# Autodesk Inventor assembly: wheel90mmwithbearing_MIR
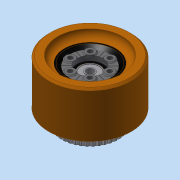
[picture p0: Inventor's stored thumbnail of the model, 180x180]
Saved by Autodesk Inventor 2014 SP1 (Build 180222100, 222)
## iProperties
Created: 2014-05-15
Part Number: wheel90mmwithbearing_MIR
Document SubType Name: Assembly
Designer: brent
Author: brent
## Documents named in this file (5)
- C:\Users\brent\Documents\electric-longboard\brent\wheel90mmwithbearing_MIR.iam
- C:\Users\brent\Documents\electric-longboard\brent\wheel90mm_MIR.ipt
- C:\Users\brent\Documents\electric-longboard\brent\608bearing_MIR.ipt
- C:\Users\brent\Documents\electric-longboard\brent\wheelinsertinner40t_MIR.ipt
- C:\Users\brent\Documents\electric-longboard\brent\wheelinsertouter_MIR.ipt
## Components (5 placed, 4 different names)
1. wheel90mm_MIR:1 — Insert:2, Insert:1, Mate:1
2. 608bearing_MIR:1 — Insert:2
3. 608bearing_MIR:2 — Insert:1
4. wheelinsertinner40t_MIR:1
5. wheelinsertouter_MIR:1 — Mate:1
## Relationships (3: Insert 2, Mate 1)
- Insert:2: wheel90mm_MIR:1 ↔ 608bearing_MIR:1
- Insert:1: wheel90mm_MIR:1 ↔ 608bearing_MIR:2
- Mate:1 (-25.4 mm): wheel90mm_MIR:1 ↔ wheelinsertouter_MIR:1
